# Autodesk Inventor assembly: Робот
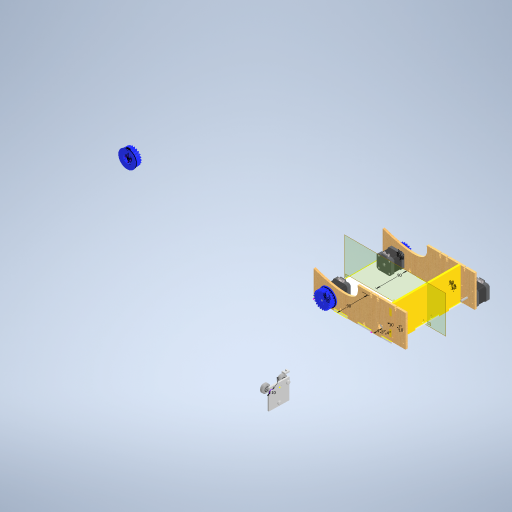
[picture p0: Inventor's stored thumbnail of the model, 512x512]
Saved by Autodesk Inventor 2024.2 (Build 282272000, 272)
## iProperties
Created: 2026-01-27
Part Number: Робот
Document SubType Name: Assembly
Designer: Service
d4: 0,000 мм
Author: Service
## Documents named in this file (9)
- C:\Users\Service\Documents\Artist-v2\3D\Робот.iam
- C:\Users\Service\Documents\Artist-v2\3D\Низ робота.ipt
- C:\Users\Service\Documents\Artist-v2\3D\бок.ipt
- C:\Users\Service\Documents\Artist-v2\3D\перед.ipt
- C:\Users\Service\Documents\Artist-v2\3D\NEMA17 42-40.ipt
- C:\Users\Service\Documents\Artist-v2\3D\Шестерня.ipt
- C:\Users\Service\Documents\крышка.ipt
- C:\Users\Service\Documents\Artist-v2\3D\каретка.iam
- C:\Users\Service\Documents\Artist-v2\3D\stl\крепеж валика.ipt
## Components (14 placed, 8 different names)
1. Низ робота:1 — Совмещение:1, Заподлицо:2, Симметрия:1, Совмещение:2, Заподлицо:3, Совмещение:3, Заподлицо:5, Совмещение:12, Заподлицо:9
2. бок:1 — Совмещение:1, Заподлицо:2, Симметрия:1, Совмещение:4, Совмещение:5, Совмещение:13, Симметрия:2
3. бок:2 — Совмещение:2, Заподлицо:3, Совмещение:6, Совмещение:7, Совмещение:8, Совмещение:10, Заподлицо:6, Совмещение:19, Совмещение:20, Совмещение:21, Совмещение:22, Совмещение:23, Заподлицо:8, Симметрия:2
4. перед:1 — Совмещение:3, Заподлицо:5, Заподлицо:7, Заподлицо:8
5. NEMA17 42-40:1 — Совмещение:4, Совмещение:5, Совмещение:12, Совмещение:14
6. NEMA17 42-40:2 — Совмещение:6, Совмещение:7, Совмещение:8, Совмещение:9
7. Шестерня:1 — Совмещение:13, Совмещение:14
8. Шестерня:2
9. Шестерня:3 — Совмещение:19, Совмещение:20
10. Шестерня:4 — Совмещение:9, Совмещение:10
11. крышка:1 — Заподлицо:6, Заподлицо:7
12. каретка:1 [sub-assembly] — Совмещение:15, Касательность:1, Касательность:2
13. NEMA17 42-40:3 — Совмещение:21, Совмещение:22, Совмещение:23
14. крепеж валика:1 — Заподлицо:9
## Relationships (30: Mate 19, Flush 7, Symmetry 2, Tangent 2)
- Совмещение:1 [Mate]: Низ робота:1 ↔ бок:1
- Заподлицо:2 [Flush]: Низ робота:1 ↔ бок:1
- Симметрия:1 [Symmetry]: Низ робота:1 ↔ бок:1
- Совмещение:2 [Mate]: Низ робота:1 ↔ бок:2
- Заподлицо:3 [Flush]: Низ робота:1 ↔ бок:2
- Совмещение:3 [Mate]: Низ робота:1 ↔ перед:1
- Заподлицо:5 [Flush]: Низ робота:1 ↔ перед:1
- Совмещение:4 [Mate]: бок:1 ↔ NEMA17 42-40:1
- Совмещение:5 [Mate]: бок:1 ↔ NEMA17 42-40:1
- Совмещение:6 [Mate]: бок:2 ↔ NEMA17 42-40:2
- Совмещение:7 [Mate]: бок:2 ↔ NEMA17 42-40:2
- Совмещение:8 [Mate]: бок:2 ↔ NEMA17 42-40:2
- Совмещение:9 [Mate]: NEMA17 42-40:2 ↔ Шестерня:4
- Совмещение:10 [Mate]: бок:2 ↔ Шестерня:4
- Совмещение:12 [Mate]: Низ робота:1 ↔ NEMA17 42-40:1
- Совмещение:13 [Mate]: бок:1 ↔ Шестерня:1
- Совмещение:14 [Mate]: NEMA17 42-40:1 ↔ Шестерня:1
- Заподлицо:6 [Flush]: бок:2 ↔ крышка:1
- Заподлицо:7 [Flush]: перед:1 ↔ крышка:1
- Совмещение:15 [Mate] (13.2 mm): каретка:1
- Касательность:1 [Tangent]: каретка:1
- Касательность:2 [Tangent]: каретка:1
- Совмещение:19 [Mate]: бок:2 ↔ Шестерня:3
- Совмещение:20 [Mate]: бок:2 ↔ Шестерня:3
- Совмещение:21 [Mate]: бок:2 ↔ NEMA17 42-40:3
- Совмещение:22 [Mate]: бок:2 ↔ NEMA17 42-40:3
- Совмещение:23 [Mate]: бок:2 ↔ NEMA17 42-40:3
- Заподлицо:8 [Flush]: бок:2 ↔ перед:1
- Симметрия:2 [Symmetry]: бок:1 ↔ бок:2
- Заподлицо:9 [Flush]: Низ робота:1 ↔ крепеж валика:1
